# Autodesk Inventor assembly: flat_assembily
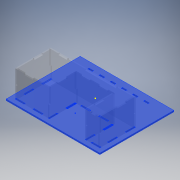
[picture p0: Inventor's stored thumbnail of the model, 180x180]
Saved by Autodesk Inventor 2017.2 (Build 212233000, 233)
## iProperties
Created: 2017-06-02
Part Number: flat_assembily
Document SubType Name: Assembly
Designer: SandeepSH
Author: SandeepSH
## Documents named in this file (9)
- C:\Users\SandeepSH\Dropbox\MSC\Project\inventor\flat_nest\flat_assembily.iam
- C:\Users\SandeepSH\Dropbox\MSC\Project\inventor\flat_nest\base.ipt
- C:\Users\SandeepSH\Dropbox\MSC\Project\inventor\flat_nest\cham_back.ipt
- C:\Users\SandeepSH\Dropbox\MSC\Project\inventor\flat_nest\cham_side.ipt
- C:\Users\SandeepSH\Dropbox\MSC\Project\inventor\flat_nest\back.ipt
- C:\Users\SandeepSH\Dropbox\MSC\Project\inventor\flat_nest\side.ipt
- C:\Users\SandeepSH\Dropbox\MSC\Project\inventor\flat_nest\front_left.ipt
- C:\Users\SandeepSH\Dropbox\MSC\Project\inventor\flat_nest\fromt_right.ipt
- C:\Users\SandeepSH\Dropbox\MSC\Project\inventor\flat_nest\top.ipt
## Components (10 placed, 8 different names)
1. base:1 — Mate:1, Mate:2, Mate:3, Mate:4, Mate:5, Mate:7, Mate:8, Mate:9, Mate:10, Mate:11, Mate:12, Mate:13, Mate:14, Mate:15, Mate:16, Mate:17
2. cham_back:1 — Mate:1, Mate:2, Mate:3, Mate:6
3. cham_side:1 — Mate:4, Mate:5
4. cham_side:2 — Mate:6, Mate:7
5. back:1 — Mate:8, Mate:9
6. side:1 — Mate:12, Mate:13
7. side:2 — Mate:10, Mate:11, Mate:18
8. front_left:1 — Mate:14, Mate:15
9. fromt_right:1 — Mate:16, Mate:17, Mate:19
10. top:1 — Mate:18, Mate:19
## Relationships (19: Mate 19)
- Mate:1: base:1 ↔ cham_back:1
- Mate:2: base:1 ↔ cham_back:1
- Mate:3: base:1 ↔ cham_back:1
- Mate:4: base:1 ↔ cham_side:1
- Mate:5: base:1 ↔ cham_side:1
- Mate:6: cham_back:1 ↔ cham_side:2
- Mate:7: base:1 ↔ cham_side:2
- Mate:8: base:1 ↔ back:1
- Mate:9: base:1 ↔ back:1
- Mate:10: base:1 ↔ side:2
- Mate:11: base:1 ↔ side:2
- Mate:12: base:1 ↔ side:1
- Mate:13: base:1 ↔ side:1
- Mate:14: base:1 ↔ front_left:1
- Mate:15: base:1 ↔ front_left:1
- Mate:16: base:1 ↔ fromt_right:1
- Mate:17: base:1 ↔ fromt_right:1
- Mate:18: side:2 ↔ top:1
- Mate:19: fromt_right:1 ↔ top:1
